# Autodesk Inventor assembly: M5 Screw with Tee Nut_MIR1
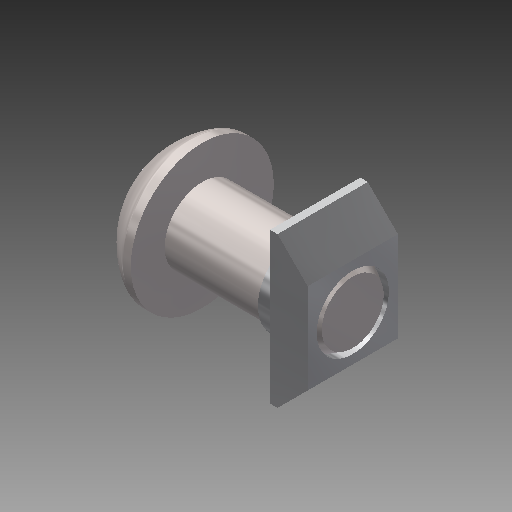
[picture p0: Inventor's stored thumbnail of the model, 512x512]
Saved by Autodesk Inventor 2017 (Build 210142000, 142)
## iProperties
Created: 2014-02-18
Part Number: M5 Screw with Tee Nut_MIR1
Document SubType Name: Assembly
Designer: umr
Mass: 2.70106 g
Surface Area: 5.57941 cm^2
Volume: 0.422368 cm^3
Density: 6.39505 g/cm^3
Author: umr
Sending System: SolidWorks 2014
Last Author: Rory
Last Saved: 2016-05-20
## Documents named in this file (3)
- D:\SeniorProject\Models2\Gantry\M5 Screw with Tee Nut_MIR1.iam
- D:\SeniorProject\Models2\Gantry\Tee Nut_MIR2.ipt
- D:\SeniorProject\Models2\Gantry\M5 Screw_MIR1.ipt
## Components (2 placed, 2 different names)
1. Tee Nut_MIR2:1 — Flush:1, Mate:2
2. M5 Screw_MIR1:1 — Flush:1, Mate:2
## Relationships (2: Flush 1, Mate 1)
- Flush:1: Tee Nut_MIR2:1 ↔ M5 Screw_MIR1:1
- Mate:2: Tee Nut_MIR2:1 ↔ M5 Screw_MIR1:1
